# Autodesk Inventor assembly: z
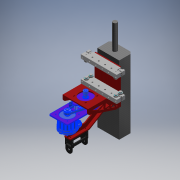
[picture p0: Inventor's stored thumbnail of the model, 180x180]
Saved by Autodesk Inventor 2019 (Build 230136000, 136)
## iProperties
Created: 2017-12-19
Part Number: z
Document SubType Name: Assembly
Designer: torba
Author: torba
## Documents named in this file (10)
- C:\Users\torba\OneDrive\Documents\Inventor\Plasma 5x10\z.iam
- C:\Users\torba\OneDrive\Documents\Inventor\Plasma 5x10\CRP102-00.ipt
- C:\Users\torba\OneDrive\Documents\Inventor\Plasma 5x10\chineese z.ipt
- C:\Users\torba\OneDrive\Documents\Inventor\Plasma 5x10\X Motor Mount.ipt
- C:\Users\torba\OneDrive\Documents\Inventor\Plasma 5x10\Z Adapter.ipt
- C:\Users\torba\OneDrive\Documents\Inventor\Plasma 5x10\Drag Chain End.ipt
- C:\Users\torba\OneDrive\Documents\Inventor\Plasma 5x10\X motor supports.ipt
- C:\Users\torba\OneDrive\Documents\Inventor\Plasma 5x10\XZ chain Support top.ipt
- C:\Users\torba\OneDrive\Documents\Inventor\Plasma 5x10\XZ chain Support.ipt
- C:\Users\torba\OneDrive\Documents\Inventor\Plasma 5x10\x reduction assembly 2.iam
## Components (11 placed, 9 different names)
1. CRP102-00:1 — Mate:1, Flush:3, Flush:4, Mate:2, Mate:10, Mate:11, Flush:8, Flush:10
2. CRP102-00:2 — Mate:2, Mate:16, Mate:17, Flush:8, Flush:10
3. chineese z:1 — Mate:1, Flush:3, Flush:4
4. X Motor Mount:1 — Mate:16, Flush:9, Mate:20, Flush:17, Mate:25, Flush:20, Mate:36
5. Z Adapter:1 — Mate:10, Mate:11, Mate:17, Flush:9, Flush:16, Mate:26, Mate:35, Mate:37
6. Drag Chain End:1 — Mate:27, Mate:28, Mate:29
7. X motor supports:1 — Flush:17, Flush:20, Mate:35, Mate:36
8. X motor supports:2 — Mate:20, Flush:16, Flush:19, Mate:37
9. XZ chain Support top:1 — Mate:22, Mate:24, Flush:18, Mate:27, Mate:28, Mate:29
10. XZ chain Support:1 — Mate:22, Mate:24, Flush:18, Mate:25, Mate:26, Flush:19
11. x reduction assembly 2:1 [sub-assembly]
## Relationships (32: Mate 21, Flush 10, Angle 1)
- Mate:1 (6.35 mm): CRP102-00:1 ↔ chineese z:1
- Flush:3 (42.4561 mm): CRP102-00:1 ↔ chineese z:1
- Flush:4 (-25.4 mm): CRP102-00:1 ↔ chineese z:1
- Mate:2 (107.95 mm): CRP102-00:1 ↔ CRP102-00:2
- Mate:10: CRP102-00:1 ↔ Z Adapter:1
- Mate:11: CRP102-00:1 ↔ Z Adapter:1
- Mate:16: CRP102-00:2 ↔ X Motor Mount:1
- Mate:17: CRP102-00:2 ↔ Z Adapter:1
- Flush:8: CRP102-00:1 ↔ CRP102-00:2
- Flush:9: X Motor Mount:1 ↔ Z Adapter:1
- Flush:10: CRP102-00:1 ↔ CRP102-00:2
- Mate:20: X Motor Mount:1 ↔ X motor supports:2
- Flush:16: Z Adapter:1 ↔ X motor supports:2
- Flush:17: X Motor Mount:1 ↔ X motor supports:1
- Mate:22: XZ chain Support top:1 ↔ XZ chain Support:1
- Mate:24: XZ chain Support top:1 ↔ XZ chain Support:1
- Flush:18 (15.875 mm): XZ chain Support top:1 ↔ XZ chain Support:1
- Mate:25: X Motor Mount:1 ↔ XZ chain Support:1
- Mate:26: Z Adapter:1 ↔ XZ chain Support:1
- Flush:19 (73.025 mm): X motor supports:2 ↔ XZ chain Support:1
- Mate:27: Drag Chain End:1 ↔ XZ chain Support top:1
- Mate:28: Drag Chain End:1 ↔ XZ chain Support top:1
- Mate:29: Drag Chain End:1 ↔ XZ chain Support top:1
- Flush:20: X Motor Mount:1 ↔ X motor supports:1
- Mate:35: Z Adapter:1 ↔ X motor supports:1
- Mate:36: X Motor Mount:1 ↔ X motor supports:1
- Mate:37: Z Adapter:1 ↔ X motor supports:2
- [Mate]: X Motor Mount:1 ↔ x reduction assembly 2:1
- [Mate]: X Motor Mount:1 ↔ x reduction assembly 2:1
- [Angle] (0 deg): X Motor Mount:1 ↔ x reduction assembly 2:1
- [Mate]: X Motor Mount:1 ↔ x reduction assembly 2:1
- [Mate]: X Motor Mount:1 ↔ x reduction assembly 2:1
